# Autodesk Inventor assembly: screej assambly
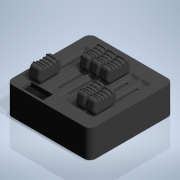
[picture p0: Inventor's stored thumbnail of the model, 180x180]
Saved by Autodesk Inventor 2022 (Build 260153000, 153)
## iProperties
Created: 2023-06-29
Part Number: screej assambly
Document SubType Name: Assembly
Designer: alex
Author: alex
## Documents named in this file (5)
- C:\Users\alex\Documents\PlatformIO\Projects\screej\Hardware\3D model\screej assambly.iam
- C:\Users\alex\Documents\PlatformIO\Projects\screej\Hardware\3D model\potknob.ipt
- C:\Users\alex\Documents\PlatformIO\Projects\screej\Hardware\3D model\potknobsmall.ipt
- C:\Users\alex\Downloads\Part8.ipt
- C:\Users\alex\Documents\PlatformIO\Projects\screej\Hardware\3D model\hardware\botom.ipt
## Components (8 placed, 4 different names)
1. potknob:1 — Mate:1
2. potknobsmall:1 — Mate:2
3. potknobsmall:2 — Mate:3
4. potknobsmall:3 — Mate:6
5. potknobsmall:4 — Mate:4
6. potknobsmall:5 — Mate:5
7. Part8:1 — Flush:1, Flush:2, Flush:3
8. botom:1 — Flush:3
## Relationships (9: Mate 6, Flush 3)
- Mate:1: potknob:1
- Mate:2: potknobsmall:1
- Mate:3: potknobsmall:2
- Mate:4: potknobsmall:4
- Mate:5: potknobsmall:5
- Mate:6: potknobsmall:3
- Flush:1: Part8:1
- Flush:2: Part8:1
- Flush:3: Part8:1 ↔ botom:1
